# Autodesk Inventor assembly: mini sumô montado
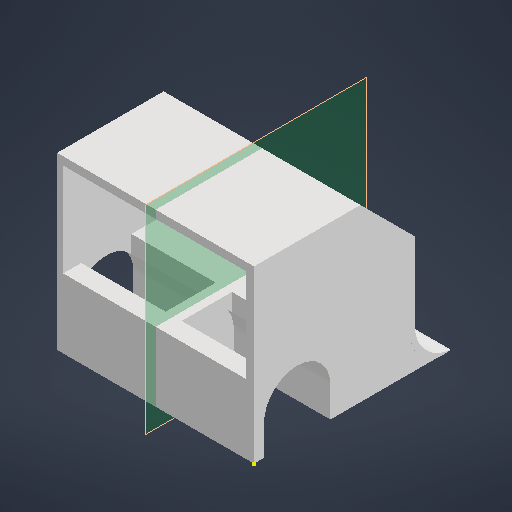
[picture p0: Inventor's stored thumbnail of the model, 512x512]
Saved by Autodesk Inventor 2026.1 (Build 301233000, 233)
## iProperties
Created: 2025-11-14
Part Number: mini sumô montado
Document SubType Name: Assembly
Designer: panto
Author: panto
## Documents named in this file (3)
- C:\Users\panto\OneDrive\Documentos\Inventor\MINI SUMÔ GEAR 2025 - EQUIPE 2\mini sumô montado.iam
- C:\Users\panto\OneDrive\Documentos\Inventor\MINI SUMÔ GEAR 2025 - EQUIPE 2\Mini sumô v3.ipt
- C:\Users\panto\OneDrive\Documentos\Inventor\MINI SUMÔ GEAR 2025 - EQUIPE 2\tampa mini sumôipt.ipt
## Components (2 placed, 2 different names)
1. Mini sumô v3:1 — Coincidente:1
2. tampa mini sumôipt:1 — Coincidente:1
## Relationships (1: Mate 1)
- Coincidente:1 [Mate]: Mini sumô v3:1 ↔ tampa mini sumôipt:1
